# Autodesk Inventor assembly: Headlight
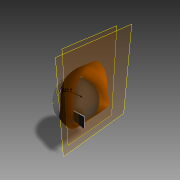
[picture p0: Inventor's stored thumbnail of the model, 180x180]
Saved by Autodesk Inventor 2016 (Build 200138000, 138)
## iProperties
Created: 2015-08-08
Part Number: Headlight
Document SubType Name: Assembly
Designer: Yann
Author: Yann
## Documents named in this file (8)
- C:\Users\Yann\Documents\GitHub\BIKAIR_CAD\Source\Front_Train\Headlight.iam
- C:\Users\Yann\Documents\GitHub\BIKAIR_CAD\Source\Front_Train\Headlight_Body.ipt
- C:\Users\Yann\Documents\GitHub\BIKAIR_CAD\Source\Front_Train\Headlight_Light.ipt
- C:\Users\Yann\Documents\GitHub\BIKAIR_CAD\Source\Front_Train\Headlight\Low_beam_optic.ipt
- C:\Users\Yann\Documents\GitHub\BIKAIR_CAD\Source\Front_Train\Headlight\12752-70239-sideemitter-rev1_Customer.ipt
- C:\Users\Yann\Documents\GitHub\BIKAIR_CAD\Source\Front_Train\Headlight\Turning_signal_optic.ipt
- C:\Users\Yann\Documents\GitHub\BIKAIR_CAD\Source\Front_Train\Headlight\Headlight_Round_Body.ipt
- C:\Users\Yann\Documents\GitHub\BIKAIR_CAD\Source\Front_Train\Headlight\Headlight_Mounting_Bracket.ipt
## Components (9 placed, 7 different names)
1. Headlight_Body:1 — Mate:1, Flush:1, Flush:2, Flush:4
2. Headlight_Light:1 — Flush:3, Flush:4
3. Low_beam_optic:1 — Mate:2
4. 12752-70239-sideemitter-rev1_Customer:1
5. Turning_signal_optic:1
6. Turning_signal_optic:2
7. Low_beam_optic:2 — Mate:3
8. Headlight_Round_Body:1 — Flush:5
9. Headlight_Mounting_Bracket:1
## Relationships (8: Flush 5, Mate 3)
- Mate:1: Headlight_Body:1
- Flush:1: Headlight_Body:1
- Flush:2: Headlight_Body:1
- Flush:3 (1.716 mm): Headlight_Light:1
- Flush:4 (117.65 mm): Headlight_Body:1 ↔ Headlight_Light:1
- Mate:2: Low_beam_optic:1
- Mate:3: Low_beam_optic:2
- Flush:5: Headlight_Round_Body:1
